# Autodesk Inventor assembly: Ensamble_completo
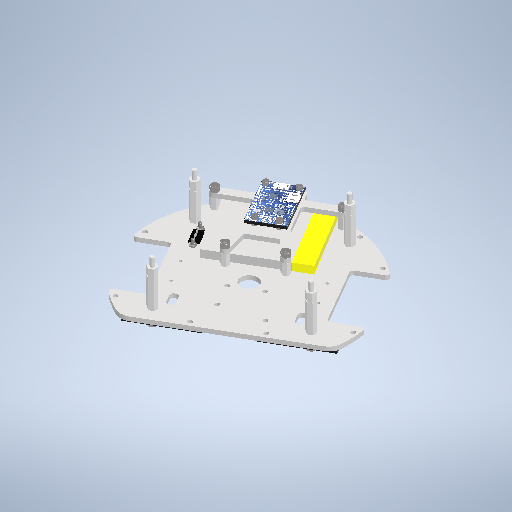
[picture p0: Inventor's stored thumbnail of the model, 512x512]
Saved by Autodesk Inventor 2025.3 (Build 293356030, 356C)
## iProperties
Created: 2025-10-21
Part Number: Ensamble_completo
Document SubType Name: Assembly
Designer: brene
Author: brene
## Documents named in this file (18)
- D:\OneDrive - Estudiantes ITCR\Documentos\GitHub\Atta-Bot-STEM\Chasis\Rediseño_Diego&Carlos\Carcasa 4.0 Rediseño\Ensamble_completo.iam
- D:\OneDrive - Estudiantes ITCR\Documentos\GitHub\Atta-Bot-STEM\Chasis\Rediseño_Diego&Carlos\Carcasa 4.0 Rediseño\base_chasis_v6\base_chasis_v4-dimsAjustadas.ipt
- D:\OneDrive - Estudiantes ITCR\Documentos\GitHub\Atta-Bot-STEM\Chasis\Rediseño_Diego&Carlos\Carcasa 4.0 Rediseño\base_chasis_v6.ipt
- D:\OneDrive - Estudiantes ITCR\Documentos\GitHub\Atta-Bot-STEM\Chasis\Rediseño_Diego&Carlos\Content Center Files\en-US\ISO 4762(2)\ISO 4762 - M2 x 12ISO.ipt
- D:\OneDrive - Estudiantes ITCR\Documentos\GitHub\Atta-Bot-STEM\Chasis\Rediseño_Diego&Carlos\switch.ipt
- D:\OneDrive - Estudiantes ITCR\Documentos\GitHub\Atta-Bot-STEM\Chasis\Rediseño_Diego&Carlos\Content Center Files\en-US\ISO 4762(2)\ISO 4762 - M2 x 8ISO.ipt
- D:\OneDrive - Estudiantes ITCR\Documentos\GitHub\Atta-Bot-STEM\Chasis\Rediseño_Diego&Carlos\Content Center Files\en-US\ISO 4032(2)\ISO 4032 - M2 - ISO.ipt
- D:\OneDrive - Estudiantes ITCR\Documentos\GitHub\Atta-Bot-STEM\Chasis\Rediseño_Diego&Carlos\ball_caster.ipt
- D:\OneDrive - Estudiantes ITCR\Documentos\GitHub\Atta-Bot-STEM\Chasis\Rediseño_Diego&Carlos\sensorInferior.ipt
- D:\OneDrive - Estudiantes ITCR\Documentos\GitHub\Atta-Bot-STEM\Chasis\Rediseño_Diego&Carlos\Content Center Files\en-US\ISO 4762(2)\ISO 4762 - M3 x 12ISO.ipt
- D:\OneDrive - Estudiantes ITCR\Documentos\GitHub\Atta-Bot-STEM\Chasis\Rediseño_Diego&Carlos\Content Center Files\en-US\ISO 4032(2)\ISO 4032 - M3 - ISO.ipt
- D:\OneDrive - Estudiantes ITCR\Documentos\GitHub\Atta-Bot-STEM\Chasis\Rediseño_Diego&Carlos\spacers\hexagonal_spacer_MF_M3_H20_HEX5.5_FTD6_MTL6.ipt
- D:\OneDrive - Estudiantes ITCR\Documentos\GitHub\Atta-Bot-STEM\Chasis\Rediseño_Diego&Carlos\spacers\hexagonal_spacer_MF_M3_H06_HEX5.5_FTD3_MTL6.ipt
- D:\OneDrive - Estudiantes ITCR\Documentos\GitHub\Atta-Bot-STEM\Chasis\Rediseño_Diego&Carlos\Content Center Files\en-US\ISO 4762(2)\ISO 4762 - M3 x 8ISO.ipt
- D:\OneDrive - Estudiantes ITCR\Documentos\GitHub\Atta-Bot-STEM\Chasis\Rediseño_Diego&Carlos\spacers\hexagonal_spacer_MF_M3_H08_HEX5_FTD4_MTL8.ipt
- D:\OneDrive - Estudiantes ITCR\Documentos\GitHub\Atta-Bot-STEM\Chasis\Rediseño_Diego&Carlos\bateria.ipt
- D:\OneDrive - Estudiantes ITCR\Documentos\GitHub\Atta-Bot-STEM\Chasis\Rediseño_Diego&Carlos\base_powerboost.ipt
- D:\OneDrive - Estudiantes ITCR\Documentos\GitHub\Atta-Bot-STEM\Chasis\Rediseño_Diego&Carlos\powerboost.ipt
## Components (52 placed, 16 different names)
1. base_chasis_v4-dimsAjustadas:2 — Mate:1, Mate:2, Mate:4, Mate:6, Insert:1, Insert:2, Mate:7, Tangent:1, Tangent:2, Mate:8, Mate:10, Tangent:3, Tangent:4, Mate:12, Mate:13, Mate:14, Mate:15, Mate:24, Mate:26, Mate:32, Mate:33, Mate:34, Mate:35, Mate:36, Mate:38, Mate:44, Mate:45, Mate:46, Mate:47, Mate:48, Mate:49, Mate:50, Mate:51, Mate:52, Mate:54, Mate:56, Mate:58, Mate:60
2. switch:1 — Mate:1, Mate:2, Mate:3, Mate:5
3. ISO 4762 M2 x 8:1 — Mate:5, Mate:6
4. ISO 4762 M2 x 8:2 — Mate:3, Mate:4
5. ISO 4032 M2:1 — Insert:1
6. ISO 4032 M2:2 — Insert:2
7. ball_caster:1 — Mate:7, Tangent:1, Tangent:2, Mate:9, Mate:11
8. ISO 4762 M2 x 8:3 — Mate:10, Mate:11, Tangent:3
9. ISO 4762 M2 x 8:4 — Mate:8, Mate:9, Tangent:4
10. sensorInferior:1 — Mate:16, Mate:17, Mate:20
11. sensorInferior:2 — Mate:18, Mate:19, Mate:22
12. ISO 4762 M3 x 12:1 — Mate:20, Mate:21, Mate:25
13. ISO 4762 M3 x 12:2 — Mate:22, Mate:23, Mate:27
14. ISO 4032 M3:1 — Mate:12, Mate:13, Mate:16, Mate:17, Mate:21
15. ISO 4032 M3:2 — Mate:14, Mate:15, Mate:18, Mate:19, Mate:23
16. hexagonal_spacer_MF_M3_H20_HEX5.5_FTD6_MTL6:1 — Mate:24, Mate:25, Mate:28, Mate:29
17. hexagonal_spacer_MF_M3_H20_HEX5.5_FTD6_MTL6:2 — Mate:26, Mate:27, Mate:30, Mate:31
18. hexagonal_spacer_MF_M3_H06_HEX5.5_FTD3_MTL6:1 — Mate:28, Mate:29
19. hexagonal_spacer_MF_M3_H06_HEX5.5_FTD3_MTL6:2 — Mate:30, Mate:31
20. hexagonal_spacer_MF_M3_H20_HEX5.5_FTD6_MTL6:3 — Mate:38, Mate:39, Mate:40, Mate:41
21. hexagonal_spacer_MF_M3_H20_HEX5.5_FTD6_MTL6:4 — Mate:36, Mate:37, Mate:42, Mate:43
22. ISO 4762 M3 x 8:1 — Mate:32, Mate:33, Mate:37
23. ISO 4762 M3 x 8:2 — Mate:34, Mate:35, Mate:39
24. hexagonal_spacer_MF_M3_H06_HEX5.5_FTD3_MTL6:3 — Mate:42, Mate:43
25. hexagonal_spacer_MF_M3_H06_HEX5.5_FTD3_MTL6:4 — Mate:40, Mate:41
26. hexagonal_spacer_MF_M3_H08_HEX5_FTD4_MTL8:1 — Mate:56, Mate:57, Mate:61
27. hexagonal_spacer_MF_M3_H08_HEX5_FTD4_MTL8:2 — Mate:58, Mate:59, Mate:88
28. hexagonal_spacer_MF_M3_H08_HEX5_FTD4_MTL8:3 — Mate:52, Mate:53, Mate:89
29. hexagonal_spacer_MF_M3_H08_HEX5_FTD4_MTL8:4 — Mate:54, Mate:55, Mate:90
30. ISO 4032 M3:3 — Mate:44, Mate:45, Mate:55
31. ISO 4032 M3:4 — Mate:46, Mate:47, Mate:53
32. ISO 4032 M3:5 — Mate:50, Mate:51, Mate:59
33. ISO 4032 M3:6 — Mate:48, Mate:49, Mate:57
34. bateria:1 — Mate:60, Mate:61
35. base_powerboost:1 — Mate:62, Mate:63, Mate:64, Mate:65, Mate:66, Mate:67, Mate:68, Mate:69, Mate:80, Mate:82, Mate:84, Mate:86, Mate:88, Mate:89, Mate:90, Mate:91, Mate:92, Mate:93, Mate:94, Mate:95, Mate:96, Mate:97, Mate:98, Mate:99
36. powerboost:1 — Mate:70, Mate:71, Mate:72, Mate:73, Mate:74, Mate:75, Mate:76, Mate:77, Mate:78, Mate:79
37. ISO 4762 M2 x 12:1 — Mate:74, Mate:75, Mate:81
38. ISO 4762 M2 x 12:2 — Mate:72, Mate:73, Mate:83
39. ISO 4762 M2 x 8:5 — Mate:78, Mate:79, Mate:85
40. ISO 4762 M2 x 8:6 — Mate:76, Mate:77, Mate:87, Mate:91
41. ISO 4032 M2:3 — Mate:68, Mate:69
42. ISO 4032 M2:4 — Mate:62, Mate:63, Mate:71
43. ISO 4032 M2:5 — Mate:66, Mate:67
44. ISO 4032 M2:6 — Mate:64, Mate:65, Mate:70
45. ISO 4032 M2:7 — Mate:82, Mate:83
46. ISO 4032 M2:8 — Mate:86, Mate:87
47. ISO 4032 M2:9 — Mate:80, Mate:81
48. ISO 4032 M2:10 — Mate:84, Mate:85
49. ISO 4762 M3 x 8:3 — Mate:98, Mate:99
50. ISO 4762 M3 x 8:4 — Mate:92, Mate:93
51. ISO 4762 M3 x 8:5 — Mate:96, Mate:97
52. ISO 4762 M3 x 8:6 — Mate:94, Mate:95
## Relationships (105: Mate 99, Tangent 4, Insert 2)
- Mate:1: base_chasis_v4-dimsAjustadas:2 ↔ switch:1
- Mate:2: base_chasis_v4-dimsAjustadas:2 ↔ switch:1
- Mate:3: switch:1 ↔ ISO 4762 M2 x 8:2
- Mate:4: base_chasis_v4-dimsAjustadas:2 ↔ ISO 4762 M2 x 8:2
- Mate:5: switch:1 ↔ ISO 4762 M2 x 8:1
- Mate:6: base_chasis_v4-dimsAjustadas:2 ↔ ISO 4762 M2 x 8:1
- Insert:1: base_chasis_v4-dimsAjustadas:2 ↔ ISO 4032 M2:1
- Insert:2: base_chasis_v4-dimsAjustadas:2 ↔ ISO 4032 M2:2
- Mate:7: base_chasis_v4-dimsAjustadas:2 ↔ ball_caster:1
- Tangent:1: base_chasis_v4-dimsAjustadas:2 ↔ ball_caster:1
- Tangent:2: base_chasis_v4-dimsAjustadas:2 ↔ ball_caster:1
- Mate:8: base_chasis_v4-dimsAjustadas:2 ↔ ISO 4762 M2 x 8:4
- Mate:9: ball_caster:1 ↔ ISO 4762 M2 x 8:4
- Mate:10: base_chasis_v4-dimsAjustadas:2 ↔ ISO 4762 M2 x 8:3
- Mate:11: ball_caster:1 ↔ ISO 4762 M2 x 8:3
- Tangent:3: base_chasis_v4-dimsAjustadas:2 ↔ ISO 4762 M2 x 8:3
- Tangent:4: base_chasis_v4-dimsAjustadas:2 ↔ ISO 4762 M2 x 8:4
- Mate:12: base_chasis_v4-dimsAjustadas:2 ↔ ISO 4032 M3:1
- Mate:13: base_chasis_v4-dimsAjustadas:2 ↔ ISO 4032 M3:1
- Mate:14: base_chasis_v4-dimsAjustadas:2 ↔ ISO 4032 M3:2
- Mate:15: base_chasis_v4-dimsAjustadas:2 ↔ ISO 4032 M3:2
- Mate:16: sensorInferior:1 ↔ ISO 4032 M3:1
- Mate:17: sensorInferior:1 ↔ ISO 4032 M3:1
- Mate:18: sensorInferior:2 ↔ ISO 4032 M3:2
- Mate:19: sensorInferior:2 ↔ ISO 4032 M3:2
- Mate:20: sensorInferior:1 ↔ ISO 4762 M3 x 12:1
- Mate:21: ISO 4762 M3 x 12:1 ↔ ISO 4032 M3:1
- Mate:22: sensorInferior:2 ↔ ISO 4762 M3 x 12:2
- Mate:23: ISO 4762 M3 x 12:2 ↔ ISO 4032 M3:2
- Mate:24: base_chasis_v4-dimsAjustadas:2 ↔ hexagonal_spacer_MF_M3_H20_HEX5.5_FTD6_MTL6:1
- Mate:25: ISO 4762 M3 x 12:1 ↔ hexagonal_spacer_MF_M3_H20_HEX5.5_FTD6_MTL6:1
- Mate:26: base_chasis_v4-dimsAjustadas:2 ↔ hexagonal_spacer_MF_M3_H20_HEX5.5_FTD6_MTL6:2
- Mate:27: ISO 4762 M3 x 12:2 ↔ hexagonal_spacer_MF_M3_H20_HEX5.5_FTD6_MTL6:2
- Mate:28: hexagonal_spacer_MF_M3_H20_HEX5.5_FTD6_MTL6:1 ↔ hexagonal_spacer_MF_M3_H06_HEX5.5_FTD3_MTL6:1
- Mate:29: hexagonal_spacer_MF_M3_H20_HEX5.5_FTD6_MTL6:1 ↔ hexagonal_spacer_MF_M3_H06_HEX5.5_FTD3_MTL6:1
- Mate:30: hexagonal_spacer_MF_M3_H20_HEX5.5_FTD6_MTL6:2 ↔ hexagonal_spacer_MF_M3_H06_HEX5.5_FTD3_MTL6:2
- Mate:31: hexagonal_spacer_MF_M3_H20_HEX5.5_FTD6_MTL6:2 ↔ hexagonal_spacer_MF_M3_H06_HEX5.5_FTD3_MTL6:2
- Mate:32: base_chasis_v4-dimsAjustadas:2 ↔ ISO 4762 M3 x 8:1
- Mate:33: base_chasis_v4-dimsAjustadas:2 ↔ ISO 4762 M3 x 8:1
- Mate:34: base_chasis_v4-dimsAjustadas:2 ↔ ISO 4762 M3 x 8:2
- Mate:35: base_chasis_v4-dimsAjustadas:2 ↔ ISO 4762 M3 x 8:2
- Mate:36: base_chasis_v4-dimsAjustadas:2 ↔ hexagonal_spacer_MF_M3_H20_HEX5.5_FTD6_MTL6:4
- Mate:37: hexagonal_spacer_MF_M3_H20_HEX5.5_FTD6_MTL6:4 ↔ ISO 4762 M3 x 8:1
- Mate:38: base_chasis_v4-dimsAjustadas:2 ↔ hexagonal_spacer_MF_M3_H20_HEX5.5_FTD6_MTL6:3
- Mate:39: hexagonal_spacer_MF_M3_H20_HEX5.5_FTD6_MTL6:3 ↔ ISO 4762 M3 x 8:2
- Mate:40: hexagonal_spacer_MF_M3_H20_HEX5.5_FTD6_MTL6:3 ↔ hexagonal_spacer_MF_M3_H06_HEX5.5_FTD3_MTL6:4
- Mate:41: hexagonal_spacer_MF_M3_H20_HEX5.5_FTD6_MTL6:3 ↔ hexagonal_spacer_MF_M3_H06_HEX5.5_FTD3_MTL6:4
- Mate:42: hexagonal_spacer_MF_M3_H20_HEX5.5_FTD6_MTL6:4 ↔ hexagonal_spacer_MF_M3_H06_HEX5.5_FTD3_MTL6:3
- Mate:43: hexagonal_spacer_MF_M3_H20_HEX5.5_FTD6_MTL6:4 ↔ hexagonal_spacer_MF_M3_H06_HEX5.5_FTD3_MTL6:3
- Mate:44: base_chasis_v4-dimsAjustadas:2 ↔ ISO 4032 M3:3
- Mate:45: base_chasis_v4-dimsAjustadas:2 ↔ ISO 4032 M3:3
- Mate:46: base_chasis_v4-dimsAjustadas:2 ↔ ISO 4032 M3:4
- Mate:47: base_chasis_v4-dimsAjustadas:2 ↔ ISO 4032 M3:4
- Mate:48: base_chasis_v4-dimsAjustadas:2 ↔ ISO 4032 M3:6
- Mate:49: base_chasis_v4-dimsAjustadas:2 ↔ ISO 4032 M3:6
- Mate:50: base_chasis_v4-dimsAjustadas:2 ↔ ISO 4032 M3:5
- Mate:51: base_chasis_v4-dimsAjustadas:2 ↔ ISO 4032 M3:5
- Mate:52: base_chasis_v4-dimsAjustadas:2 ↔ hexagonal_spacer_MF_M3_H08_HEX5_FTD4_MTL8:3
- Mate:53: hexagonal_spacer_MF_M3_H08_HEX5_FTD4_MTL8:3 ↔ ISO 4032 M3:4
- Mate:54: base_chasis_v4-dimsAjustadas:2 ↔ hexagonal_spacer_MF_M3_H08_HEX5_FTD4_MTL8:4
- Mate:55: hexagonal_spacer_MF_M3_H08_HEX5_FTD4_MTL8:4 ↔ ISO 4032 M3:3
- Mate:56: base_chasis_v4-dimsAjustadas:2 ↔ hexagonal_spacer_MF_M3_H08_HEX5_FTD4_MTL8:1
- Mate:57: hexagonal_spacer_MF_M3_H08_HEX5_FTD4_MTL8:1 ↔ ISO 4032 M3:6
- Mate:58: base_chasis_v4-dimsAjustadas:2 ↔ hexagonal_spacer_MF_M3_H08_HEX5_FTD4_MTL8:2
- Mate:59: hexagonal_spacer_MF_M3_H08_HEX5_FTD4_MTL8:2 ↔ ISO 4032 M3:5
- Mate:60: base_chasis_v4-dimsAjustadas:2 ↔ bateria:1
- Mate:61: hexagonal_spacer_MF_M3_H08_HEX5_FTD4_MTL8:1 ↔ bateria:1
- Mate:62: base_powerboost:1 ↔ ISO 4032 M2:4
- Mate:63: base_powerboost:1 ↔ ISO 4032 M2:4
- Mate:64: base_powerboost:1 ↔ ISO 4032 M2:6
- Mate:65: base_powerboost:1 ↔ ISO 4032 M2:6
- Mate:66: base_powerboost:1 ↔ ISO 4032 M2:5
- Mate:67: base_powerboost:1 ↔ ISO 4032 M2:5
- Mate:68: base_powerboost:1 ↔ ISO 4032 M2:3
- Mate:69: base_powerboost:1 ↔ ISO 4032 M2:3
- Mate:70: powerboost:1 ↔ ISO 4032 M2:6
- Mate:71: powerboost:1 ↔ ISO 4032 M2:4
- Mate:72: powerboost:1 ↔ ISO 4762 M2 x 12:2
- Mate:73: powerboost:1 ↔ ISO 4762 M2 x 12:2
- Mate:74: powerboost:1 ↔ ISO 4762 M2 x 12:1
- Mate:75: powerboost:1 ↔ ISO 4762 M2 x 12:1
- Mate:76: powerboost:1 ↔ ISO 4762 M2 x 8:6
- Mate:77: powerboost:1 ↔ ISO 4762 M2 x 8:6
- Mate:78: powerboost:1 ↔ ISO 4762 M2 x 8:5
- Mate:79: powerboost:1 ↔ ISO 4762 M2 x 8:5
- Mate:80: base_powerboost:1 ↔ ISO 4032 M2:9
- Mate:81: ISO 4762 M2 x 12:1 ↔ ISO 4032 M2:9
- Mate:82: base_powerboost:1 ↔ ISO 4032 M2:7
- Mate:83: ISO 4762 M2 x 12:2 ↔ ISO 4032 M2:7
- Mate:84: base_powerboost:1 ↔ ISO 4032 M2:10
- Mate:85: ISO 4762 M2 x 8:5 ↔ ISO 4032 M2:10
- Mate:86: base_powerboost:1 ↔ ISO 4032 M2:8
- Mate:87: ISO 4762 M2 x 8:6 ↔ ISO 4032 M2:8
- Mate:88: hexagonal_spacer_MF_M3_H08_HEX5_FTD4_MTL8:2 ↔ base_powerboost:1
- Mate:89: hexagonal_spacer_MF_M3_H08_HEX5_FTD4_MTL8:3 ↔ base_powerboost:1
- Mate:90: hexagonal_spacer_MF_M3_H08_HEX5_FTD4_MTL8:4 ↔ base_powerboost:1
- Mate:91: base_powerboost:1 ↔ ISO 4762 M2 x 8:6
- Mate:92: base_powerboost:1 ↔ ISO 4762 M3 x 8:4
- Mate:93: base_powerboost:1 ↔ ISO 4762 M3 x 8:4
- Mate:94: base_powerboost:1 ↔ ISO 4762 M3 x 8:6
- Mate:95: base_powerboost:1 ↔ ISO 4762 M3 x 8:6
- Mate:96: base_powerboost:1 ↔ ISO 4762 M3 x 8:5
- Mate:97: base_powerboost:1 ↔ ISO 4762 M3 x 8:5
- Mate:98: base_powerboost:1 ↔ ISO 4762 M3 x 8:3
- Mate:99: base_powerboost:1 ↔ ISO 4762 M3 x 8:3
